# Autodesk Inventor assembly: Left Wheel
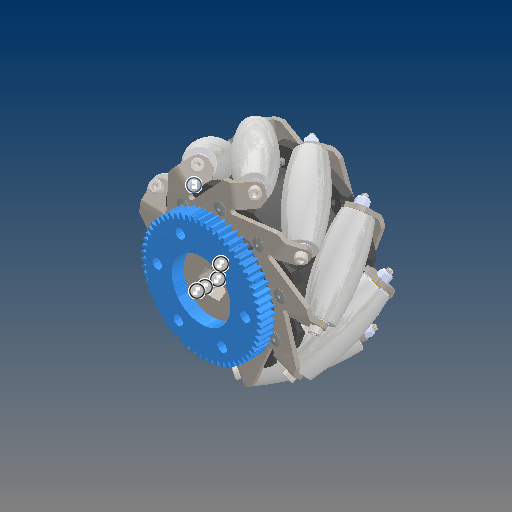
[picture p0: Inventor's stored thumbnail of the model, 512x512]
Saved by Autodesk Inventor 2024.2 (Build 282272000, 272)
## iProperties
Created: 2022-10-15
Part Number: Left Wheel
Document SubType Name: Assembly
Designer: Jason
Author: Jason
## Documents named in this file (4)
- C:\Users\alniles07\Documents\Github\8400_2024_CAD\Left Wheel - Back.iam
- C:\Users\alniles07\Documents\Github\8400_2024_CAD\Wheel Bearing.ipt
- C:\Users\alniles07\Documents\Github\8400_2024_CAD\FTC Wheel Gear.ipt
- C:\Users\alniles07\Documents\Github\8400_2024_CAD\Right Wheel.ipt
## Components (4 placed, 3 different names)
1. Right Wheel:1 — Mate:1, Mate:2, Mate:3, Mate:4, Mate:5, Mate:6, Mate:7
2. Wheel Bearing:3 — Mate:3, Mate:4
3. Wheel Bearing:4 — Mate:5, Mate:6
4. Spur Gear2:2 — Mate:1, Mate:2, Mate:7
## Relationships (7: Mate 7)
- Mate:1: Right Wheel:1 ↔ Spur Gear2:2
- Mate:2: Right Wheel:1 ↔ Spur Gear2:2
- Mate:3: Right Wheel:1 ↔ Wheel Bearing:3
- Mate:4: Right Wheel:1 ↔ Wheel Bearing:3
- Mate:5: Right Wheel:1 ↔ Wheel Bearing:4
- Mate:6: Right Wheel:1 ↔ Wheel Bearing:4
- Mate:7: Right Wheel:1 ↔ Spur Gear2:2
